# Autodesk Inventor assembly: vexGripperAssembly
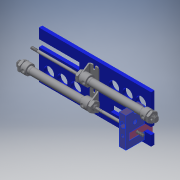
[picture p0: Inventor's stored thumbnail of the model, 180x180]
Saved by Autodesk Inventor 2016 SP1 (Build 200210100, 210)
## iProperties
Created: 2015-11-23
Part Number: vexGripperAssembly
Document SubType Name: Assembly
Designer: steele
Author: steele
## Documents named in this file (6)
- C:\snobotics\CAD-Development\robSteele\SnoBoticsSummer2015\Gripper\vexGripperAssembly.iam
- C:\snobotics\CAD-Development\robSteele\SnoBoticsSummer2015\Gripper\vexPlate.ipt
- C:\snobotics\CAD-MfgResources\McMaster-Carr\Air Cylinder\Universal Mount\Double Acting\4 in Stroke\4952K126.ipt
- C:\snobotics\CAD-MfgResources\McMaster-Carr\Air Cylinder\Universal Mount\Double Acting\3 in Stroke\6498K605.ipt
- C:\snobotics\CAD-Development\robSteele\SnoBoticsSummer2015\Gripper\vexSupportForArm.ipt
- C:\snobotics\CAD-Development\robSteele\SnoBoticsSummer2015\Gripper\vexOverSupportForArm.ipt
## Components (7 placed, 5 different names)
1. vexPlate:1 — Mate:1, Insert:1, Insert:2, Insert:3, Insert:4, Mate:2
2. 4952K126:1 — Mate:1, Insert:1, Insert:2, Insert:5
3. 4952K126:2 — Insert:3, Insert:4, Insert:6
4. 6498K605:1 — Insert:5
5. 6498K605:2 — Insert:6, Insert:7
6. vexSupportForArm:1 — Insert:7, Mate:2, Insert:8, Flush:1
7. vexOverSupportForArm:1 — Insert:8, Flush:1
## Relationships (11: Insert 8, Mate 2, Flush 1)
- Mate:1: vexPlate:1 ↔ 4952K126:1
- Insert:1: vexPlate:1 ↔ 4952K126:1
- Insert:2: vexPlate:1 ↔ 4952K126:1
- Insert:3: vexPlate:1 ↔ 4952K126:2
- Insert:4: vexPlate:1 ↔ 4952K126:2
- Insert:5: 4952K126:1 ↔ 6498K605:1
- Insert:6: 4952K126:2 ↔ 6498K605:2
- Insert:7 (-25.4 mm): 6498K605:2 ↔ vexSupportForArm:1
- Mate:2: vexPlate:1 ↔ vexSupportForArm:1
- Insert:8: vexSupportForArm:1 ↔ vexOverSupportForArm:1
- Flush:1: vexSupportForArm:1 ↔ vexOverSupportForArm:1
